# Autodesk Inventor assembly: lasermini
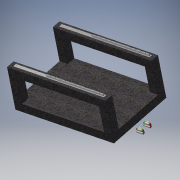
[picture p0: Inventor's stored thumbnail of the model, 180x180]
Saved by Autodesk Inventor 2016 (Build 200138000, 138)
## iProperties
Created: 2015-08-15
Part Number: lasermini
Document SubType Name: Assembly
Designer: myhome
Author: myhome
## Documents named in this file (4)
- C:\Users\myhome\Documents\Inventor\lasercad\lasermini.iam
- C:\Users\myhome\Documents\Inventor\lasercad\EpoxyGraniteBase\BaseMini.iam
- C:\Users\myhome\Documents\Inventor\lasercad\LinearGuide\HGR20\Rail-HGR20R01171-20_0.ipt
- C:\Users\myhome\Documents\Inventor\lasercad\LinearGuide\HGR20\Block-HGW20CCZ0C.iam
## Components (5 placed, 3 different names)
1. BaseMini:1 [sub-assembly] — Rotational:1, Rotational:2
2. Rail-HGR20R01171-20_0:1 — Rotational:1
3. Block-HGW20CCZ0C:1 [sub-assembly]
4. Block-HGW20CCZ0C:2 [sub-assembly]
5. Rail-HGR20R01171-20_0:2 — Rotational:2
## Relationships (2: RevoluteJoint 2)
- Rotational:1 [RevoluteJoint]: BaseMini:1 ↔ Rail-HGR20R01171-20_0:1
- Rotational:2 [RevoluteJoint]: BaseMini:1 ↔ Rail-HGR20R01171-20_0:2
